# Autodesk Inventor assembly: R-SO v11
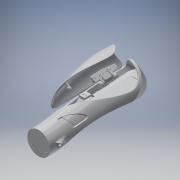
[picture p0: Inventor's stored thumbnail of the model, 180x180]
Saved by Autodesk Inventor 2018.1 (Build 221171000, 171)
## iProperties
Created: 2017-09-22
Part Number: R-SO v11
Material: 一般
Document SubType Name: Assembly
Designer: sktom
Author: sktom
## Documents named in this file (9)
- D:\CloudStrage\NextCloud\Cad_mechanical\HACKberry_SizeM\3Dmodel\R\M-R-SO\M-R-SO.iam
- D:\CloudStrage\NextCloud\Cad_mechanical\HACKberry_SizeM\3Dmodel\R\M-R-SO\M-R-SO-02.ipt
- D:\CloudStrage\NextCloud\Cad_mechanical\HACKberry_SizeM\3Dmodel\R\M-R-SO\M-R-SO-01.ipt
- D:\CloudStrage\NextCloud\Cad_mechanical\HACKberry_SizeM\3Dmodel\R\M-R-SO\M-R-SO-05.ipt
- D:\CloudStrage\NextCloud\Cad_mechanical\HACKberry_SizeM\3Dmodel\R\M-R-SO\M-R-SO-06.ipt
- D:\CloudStrage\NextCloud\Cad_mechanical\HACKberry_SizeM\3Dmodel\R\M-R-SO\M-R-SO-07.ipt
- D:\CloudStrage\NextCloud\Cad_mechanical\HACKberry_SizeM\3Dmodel\R\M-R-SO\M-R-SO-08.ipt
- D:\CloudStrage\NextCloud\Cad_mechanical\HACKberry_SizeM\3Dmodel\R\M-R-SO\M-R-SO-09.ipt
- D:\CloudStrage\NextCloud\Cad_mechanical\HACKberry_SizeM\3Dmodel\R\M-R-SO\M-R-SO-10.ipt
## Components (8 placed, 8 different names)
1. R-SO-02 v2:1 — リジッド:2
2. R-SO-01 v2:1 — リジッド:2, 挿入:7
3. R-SO-05 v2:1
4. R-SO-06 v2:1
5. R-SO-07 v2:1 — 挿入:1, 挿入:2, 挿入:3, 挿入:4, 挿入:5, 挿入:6, 挿入:7
6. R-SO-08 v2:1 — 挿入:5, 挿入:6
7. R-SO-09 v2:1 — 挿入:1, 挿入:2
8. R-SO-10 v2:1 — 挿入:3, 挿入:4
## Relationships (8: Insert 7, WeldJoint 1)
- リジッド:2 [WeldJoint] (-0.14 mm): R-SO-02 v2:1 ↔ R-SO-01 v2:1
- 挿入:1 [Insert]: R-SO-07 v2:1 ↔ R-SO-09 v2:1
- 挿入:2 [Insert]: R-SO-07 v2:1 ↔ R-SO-09 v2:1
- 挿入:3 [Insert]: R-SO-07 v2:1 ↔ R-SO-10 v2:1
- 挿入:4 [Insert]: R-SO-07 v2:1 ↔ R-SO-10 v2:1
- 挿入:5 [Insert]: R-SO-07 v2:1 ↔ R-SO-08 v2:1
- 挿入:6 [Insert]: R-SO-07 v2:1 ↔ R-SO-08 v2:1
- 挿入:7 [Insert] (0.2 mm): R-SO-01 v2:1 ↔ R-SO-07 v2:1
